# Autodesk Inventor assembly: Planetery Gear
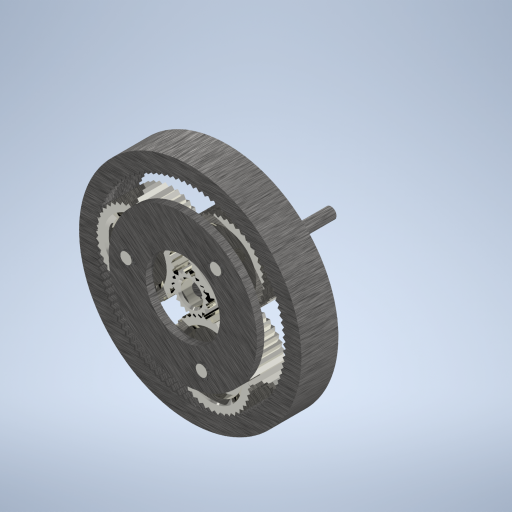
[picture p0: Inventor's stored thumbnail of the model, 512x512]
Saved by Autodesk Inventor 2024 (Build 280153000, 153)
## iProperties
Created: 2023-06-26
Part Number: Planetery Gear
Document SubType Name: Assembly
Designer: 69
Author: 69
## Documents named in this file (8)
- C:\Users\69\Desktop\git new\Planetery Gear\Planetery Gear.iam
- C:\Users\69\Desktop\git new\Planetery Gear\Ring Gear.ipt
- C:\Users\69\Desktop\git new\Planetery Gear\Sun Gear.ipt
- C:\Users\69\Desktop\git new\Planetery Gear\Planet Gear.ipt
- C:\Users\69\Desktop\git new\Planetery Gear\Carrier.ipt
- C:\Users\69\Desktop\git new\Planetery Gear\Planet Gear Shaft.ipt
- C:\Users\69\Desktop\git new\Planetery Gear\Snap Ring.ipt
- C:\Users\69\Desktop\git new\Planetery Gear\Sun Gear Shaft.ipt
## Components (13 placed, 7 different names)
1. Ring Gear:1 — Mate:1, Mate:2
2. Sun Gear:1 — Mate:6, Mate:7, Mate:10, Mate:11, Flush:1
3. Planet Gear:1 — Mate:3, Mate:8
4. Carrier:1 — Mate:1, Mate:2, Mate:3, Mate:4, Mate:6, Mate:7, Mate:12, Mate:13, Mate:14, Mate:15
5. Planet Gear Shaft:1 — Mate:4, Mate:5, Mate:8, Mate:9
6. Snap Ring:1 — Mate:5, Mate:9
7. Sun Gear Shaft:1 — Mate:10, Mate:11, Flush:1
8. Planet Gear:2 — Mate:12, Mate:16
9. Planet Gear:3 — Mate:13, Mate:17
10. Planet Gear Shaft:2 — Mate:14, Mate:17, Mate:18, Mate:21
11. Planet Gear Shaft:3 — Mate:15, Mate:16, Mate:19, Mate:20
12. Snap Ring:2 — Mate:18, Mate:21
13. Snap Ring:3 — Mate:19, Mate:20
## Relationships (22: Mate 21, Flush 1)
- Mate:1: Ring Gear:1 ↔ Carrier:1
- Mate:2: Ring Gear:1 ↔ Carrier:1
- Mate:3: Planet Gear:1 ↔ Carrier:1
- Mate:4: Carrier:1 ↔ Planet Gear Shaft:1
- Mate:5: Planet Gear Shaft:1 ↔ Snap Ring:1
- Mate:6: Sun Gear:1 ↔ Carrier:1
- Mate:7: Sun Gear:1 ↔ Carrier:1
- Mate:8: Planet Gear:1 ↔ Planet Gear Shaft:1
- Mate:9: Planet Gear Shaft:1 ↔ Snap Ring:1
- Mate:10: Sun Gear:1 ↔ Sun Gear Shaft:1
- Mate:11: Sun Gear:1 ↔ Sun Gear Shaft:1
- Flush:1: Sun Gear:1 ↔ Sun Gear Shaft:1
- Mate:12: Carrier:1 ↔ Planet Gear:2
- Mate:13: Carrier:1 ↔ Planet Gear:3
- Mate:14: Carrier:1 ↔ Planet Gear Shaft:2
- Mate:15: Carrier:1 ↔ Planet Gear Shaft:3
- Mate:16: Planet Gear:2 ↔ Planet Gear Shaft:3
- Mate:17: Planet Gear:3 ↔ Planet Gear Shaft:2
- Mate:18: Planet Gear Shaft:2 ↔ Snap Ring:2
- Mate:19: Planet Gear Shaft:3 ↔ Snap Ring:3
- Mate:20: Planet Gear Shaft:3 ↔ Snap Ring:3
- Mate:21: Planet Gear Shaft:2 ↔ Snap Ring:2
